# Autodesk Inventor assembly: ASY PRS 9500 inlet pipe
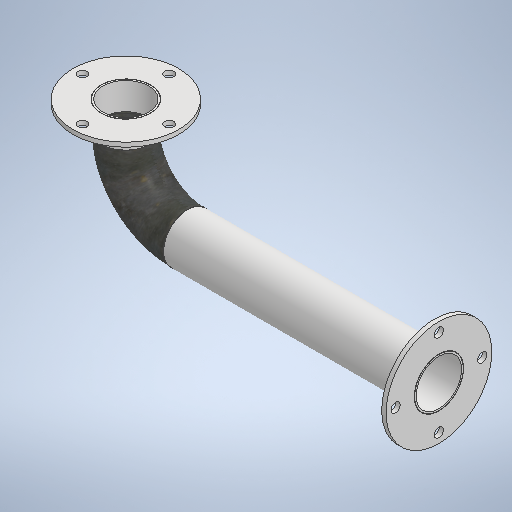
[picture p0: Inventor's stored thumbnail of the model, 512x512]
Saved by Autodesk Inventor 2026.2 (Build 302298000, 298)
## iProperties
Created: 2026-06-18
Part Number: ASY PRS 9500 inlet pipe
Document SubType Name: Assembly
Designer: admin
Author: admin
## Documents named in this file (5)
- C:\Users\admin\Documents\Inventor\PRS-Purovsk\ASY PRS 9500 inlet pipe.iam
- C:\Users\admin\Documents\Inventor\PRS-Purovsk\PRS 1633 charging blind flange_D1200 940.ipt
- C:\Users\admin\Documents\Inventor\PRS-Purovsk\PRS 9615 FDS tube 5_D1200 940.ipt
- C:\Users\admin\Documents\Inventor\PRS-Purovsk\PRS 9612 FDS tube 2_D1200 940.ipt
- C:\Users\admin\Documents\Inventor\SLM-Salemal\cc\JIS B 2312 90 Deg Long Elbow Steel 80A x Sch 40.ipt
## Components (5 placed, 4 different names)
1. PRS 1633 charging blind flange_D1200 940:1
2. PRS 1633 charging blind flange_D1200 940:2
3. PRS 9615 FDS tube 5_D1200 940:1
4. PRS 9612 FDS tube 2_D1200 940:1
5. JIS B 2312 90 Deg Long Elbow Steel 80A x Sch 40:1
## Relationships (4: WeldJoint 4)
- [WeldJoint]: PRS 1633 charging blind flange_D1200 940:2 ↔ PRS 9612 FDS tube 2_D1200 940:1
- [WeldJoint]: PRS 9612 FDS tube 2_D1200 940:1 ↔ JIS B 2312 90 Deg Long Elbow Steel 80A x Sch 40:1
- [WeldJoint]: PRS 9615 FDS tube 5_D1200 940:1 ↔ JIS B 2312 90 Deg Long Elbow Steel 80A x Sch 40:1
- [WeldJoint]: PRS 1633 charging blind flange_D1200 940:1 ↔ PRS 9615 FDS tube 5_D1200 940:1
